# Autodesk Inventor assembly: Rover
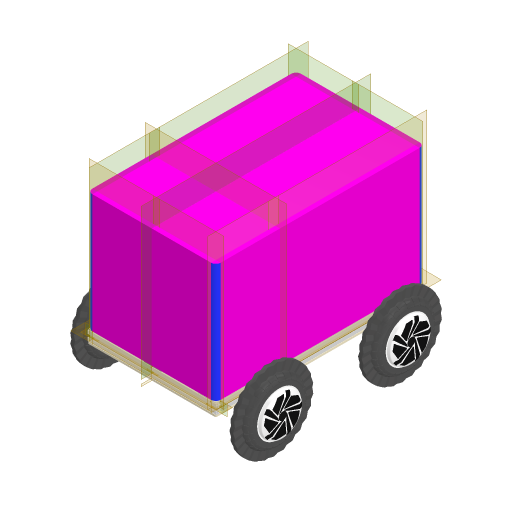
[picture p0: Inventor's stored thumbnail of the model, 512x512]
Saved by Autodesk Inventor 2023.2 (Build 272271030, 271C)
## iProperties
Created: 2024-10-30
Part Number: Rover
Document SubType Name: Assembly
Designer: I9232
Author: I9232
## Documents named in this file (10)
- D:\!Rover\Rover\Rover_construction\Rover.iam
- D:\!Rover\Rover\Rover_construction\platform.ipt
- D:\!Rover\Rover\Rover_construction\Motor, BLDC, Hoverboard Wheel, 8.0in.ipt
- D:\!Rover\Rover\Rover_construction\Profil 20x20.ipt
- D:\!Rover\Rover\Rover_construction\Крепление мотора.iam
- D:\!Rover\Rover\Rover_construction\Copter.ipt
- D:\!Rover\Rover\Rover_construction\Korpus.ipt
- D:\!Rover\Rover\Rover_construction\Уголок для профиля.ipt
- D:\!Rover\Rover\Rover_construction\Профиль 30x30\Профиль 30x30.ipt
- D:\!Rover\Rover\Rover_construction\Т-образный соединитель\Т-образный соединитель.ipt
## Components (33 placed, 10 different names)
1. platform:1 — Совмещение:1, Совмещение:2, Совмещение:107, Совмещение:119, Совмещение:120, Совмещение:121, Совмещение:169, Заподлицо:1, Заподлицо:2, Совмещение:170, Совмещение:171, Совмещение:172, Заподлицо:3, Заподлицо:4, Заподлицо:5, Заподлицо:6, Совмещение:180, Заподлицо:11
2. Copter:1
3. Корпус:1 — Совмещение:168
4. Profil 20x20:4 — Совмещение:149, Совмещение:167
5. Profil 20x20:5 — Совмещение:151, Совмещение:166
6. Profil 20x20:6 — Совмещение:152, Совмещение:165
7. Profil 20x20:7 — Совмещение:154, Совмещение:164
8. Profil 20x20:8 — Совмещение:150, Совмещение:166
9. Profil 20x20:9 — Совмещение:148, Совмещение:167
10. Profil 20x20:10 — Совмещение:153, Совмещение:165
11. Profil 20x20:11 — Совмещение:155, Совмещение:164
12. Т-образный соединитель:1 — Заподлицо:21, Совмещение:186, Совмещение:188
13. Т-образный соединитель:2 — Заподлицо:22, Совмещение:187, Заподлицо:23
14. Мотор гироскутера — Совмещение:122, Совмещение:123, Совмещение:124
15. Motor, BLDC, Hoverboard Wheel, 8.0in:4 — Совмещение:116, Совмещение:117, Совмещение:118
16. Motor, BLDC, Hoverboard Wheel, 8.0in:5 — Совмещение:112, Совмещение:113, Совмещение:115
17. Motor, BLDC, Hoverboard Wheel, 8.0in:6 — Совмещение:110, Совмещение:111, Совмещение:114
18. Profil 20x20:1 — Симметрия:3, Заподлицо:14, Совмещение:184, Заподлицо:18, Совмещение:185
19. Profil 20x20:2 — Симметрия:3, Заподлицо:12, Совмещение:181, Заподлицо:13, Заподлицо:20
20. Profil 20x20:3 — Заподлицо:18
21. Профиль 30x30:5 — Совмещение:179, Совмещение:180, Заподлицо:11, Заподлицо:21, Заподлицо:23
22. Профиль 30x30:2 — Совмещение:171, Совмещение:173, Заподлицо:3, Заподлицо:7, Заподлицо:10, Заподлицо:12, Совмещение:181, Совмещение:182, Совмещение:183
23. Профиль 30x30:3 — Совмещение:170, Заподлицо:5, Заподлицо:6, Совмещение:175, Совмещение:176, Совмещение:186, Совмещение:188
24. Профиль 30x30:4 — Совмещение:172, Совмещение:174, Заподлицо:4, Совмещение:177, Совмещение:178, Заподлицо:13, Заподлицо:14, Совмещение:184, Заподлицо:17, Заподлицо:19
25. Профиль 30x30:1 — Совмещение:169, Заподлицо:1, Заподлицо:2, Совмещение:173, Совмещение:174, Заподлицо:8, Заподлицо:9, Совмещение:179, Заподлицо:22, Совмещение:187
26. Крепление мотора:1 [sub-assembly] — Совмещение:116, Совмещение:117, Совмещение:118, Совмещение:119, Симметрия:2, Совмещение:152, Совмещение:153, Совмещение:183
27. Крепление мотора:2 [sub-assembly] — Совмещение:107, Совмещение:122, Совмещение:123, Совмещение:124, Симметрия:2, Совмещение:150, Совмещение:151, Заподлицо:19, Совмещение:185
28. Крепление мотора:3 [sub-assembly] — Совмещение:110, Совмещение:111, Совмещение:114, Совмещение:121, Симметрия:1, Совмещение:154, Совмещение:155, Совмещение:182, Заподлицо:20
29. Крепление мотора:4 [sub-assembly] — Совмещение:112, Совмещение:113, Совмещение:115, Совмещение:120, Симметрия:1, Совмещение:148, Совмещение:149, Заподлицо:17
30. Уголок для профиля:1 — Заподлицо:8, Совмещение:178
31. Уголок для профиля:2 — Совмещение:175, Заподлицо:7
32. Уголок для профиля:3 — Совмещение:168, Заподлицо:9, Заподлицо:10
33. Уголок для профиля:4 — Совмещение:176, Совмещение:177
## Relationships (75: Mate 51, Flush 21, Symmetry 3)
- Совмещение:1 [Mate]: platform:1
- Совмещение:2 [Mate]: platform:1
- Совмещение:107 [Mate]: platform:1 ↔ Крепление мотора:2
- Совмещение:110 [Mate]: Motor, BLDC, Hoverboard Wheel, 8.0in:6 ↔ Крепление мотора:3
- Совмещение:111 [Mate]: Motor, BLDC, Hoverboard Wheel, 8.0in:6 ↔ Крепление мотора:3
- Совмещение:112 [Mate]: Motor, BLDC, Hoverboard Wheel, 8.0in:5 ↔ Крепление мотора:4
- Совмещение:113 [Mate]: Motor, BLDC, Hoverboard Wheel, 8.0in:5 ↔ Крепление мотора:4
- Совмещение:114 [Mate]: Motor, BLDC, Hoverboard Wheel, 8.0in:6 ↔ Крепление мотора:3
- Совмещение:115 [Mate]: Motor, BLDC, Hoverboard Wheel, 8.0in:5 ↔ Крепление мотора:4
- Совмещение:116 [Mate]: Motor, BLDC, Hoverboard Wheel, 8.0in:4 ↔ Крепление мотора:1
- Совмещение:117 [Mate]: Motor, BLDC, Hoverboard Wheel, 8.0in:4 ↔ Крепление мотора:1
- Совмещение:118 [Mate]: Motor, BLDC, Hoverboard Wheel, 8.0in:4 ↔ Крепление мотора:1
- Совмещение:119 [Mate]: platform:1 ↔ Крепление мотора:1
- Совмещение:120 [Mate]: platform:1 ↔ Крепление мотора:4
- Совмещение:121 [Mate]: platform:1 ↔ Крепление мотора:3
- Совмещение:122 [Mate]: Мотор гироскутера ↔ Крепление мотора:2
- Совмещение:123 [Mate]: Мотор гироскутера ↔ Крепление мотора:2
- Совмещение:124 [Mate]: Мотор гироскутера ↔ Крепление мотора:2
- Симметрия:1 [Symmetry]: Крепление мотора:3 ↔ Крепление мотора:4
- Симметрия:2 [Symmetry]: Крепление мотора:1 ↔ Крепление мотора:2
- Симметрия:3 [Symmetry]: Profil 20x20:1 ↔ Profil 20x20:2
- Совмещение:148 [Mate]: Profil 20x20:9 ↔ Крепление мотора:4
- Совмещение:149 [Mate]: Profil 20x20:4 ↔ Крепление мотора:4
- Совмещение:150 [Mate]: Profil 20x20:8 ↔ Крепление мотора:2
- Совмещение:151 [Mate]: Profil 20x20:5 ↔ Крепление мотора:2
- Совмещение:152 [Mate]: Profil 20x20:6 ↔ Крепление мотора:1
- Совмещение:153 [Mate]: Profil 20x20:10 ↔ Крепление мотора:1
- Совмещение:154 [Mate]: Profil 20x20:7 ↔ Крепление мотора:3
- Совмещение:155 [Mate]: Profil 20x20:11 ↔ Крепление мотора:3
- Совмещение:164 [Mate] (30 mm): Profil 20x20:7 ↔ Profil 20x20:11
- Совмещение:165 [Mate] (30 mm): Profil 20x20:6 ↔ Profil 20x20:10
- Совмещение:166 [Mate] (30 mm): Profil 20x20:5 ↔ Profil 20x20:8
- Совмещение:167 [Mate] (30 mm): Profil 20x20:4 ↔ Profil 20x20:9
- Совмещение:168 [Mate]: Корпус:1 ↔ Уголок для профиля:3
- Совмещение:169 [Mate]: platform:1 ↔ Профиль 30x30:1
- Заподлицо:1 [Flush]: platform:1 ↔ Профиль 30x30:1
- Заподлицо:2 [Flush]: platform:1 ↔ Профиль 30x30:1
- Совмещение:170 [Mate]: platform:1 ↔ Профиль 30x30:3
- Совмещение:171 [Mate]: platform:1 ↔ Профиль 30x30:2
- Совмещение:172 [Mate]: platform:1 ↔ Профиль 30x30:4
- Совмещение:173 [Mate]: Профиль 30x30:2 ↔ Профиль 30x30:1
- Заподлицо:3 [Flush]: platform:1 ↔ Профиль 30x30:2
- Совмещение:174 [Mate]: Профиль 30x30:4 ↔ Профиль 30x30:1
- Заподлицо:4 [Flush]: platform:1 ↔ Профиль 30x30:4
- Заподлицо:5 [Flush]: platform:1 ↔ Профиль 30x30:3
- Заподлицо:6 [Flush]: platform:1 ↔ Профиль 30x30:3
- Совмещение:175 [Mate]: Профиль 30x30:3 ↔ Уголок для профиля:2
- Заподлицо:7 [Flush]: Профиль 30x30:2 ↔ Уголок для профиля:2
- Совмещение:176 [Mate]: Профиль 30x30:3 ↔ Уголок для профиля:4
- Совмещение:177 [Mate]: Профиль 30x30:4 ↔ Уголок для профиля:4
- Заподлицо:8 [Flush]: Профиль 30x30:1 ↔ Уголок для профиля:1
- Совмещение:178 [Mate]: Профиль 30x30:4 ↔ Уголок для профиля:1
- Заподлицо:9 [Flush]: Профиль 30x30:1 ↔ Уголок для профиля:3
- Заподлицо:10 [Flush]: Профиль 30x30:2 ↔ Уголок для профиля:3
- Совмещение:179 [Mate]: Профиль 30x30:5 ↔ Профиль 30x30:1
- Совмещение:180 [Mate]: platform:1 ↔ Профиль 30x30:5
- Заподлицо:11 [Flush]: platform:1 ↔ Профиль 30x30:5
- Заподлицо:12 [Flush]: Profil 20x20:2 ↔ Профиль 30x30:2
- Совмещение:181 [Mate]: Profil 20x20:2 ↔ Профиль 30x30:2
- Заподлицо:13 [Flush]: Profil 20x20:2 ↔ Профиль 30x30:4
- Совмещение:182 [Mate]: Профиль 30x30:2 ↔ Крепление мотора:3
- Совмещение:183 [Mate]: Профиль 30x30:2 ↔ Крепление мотора:1
- Заподлицо:14 [Flush]: Profil 20x20:1 ↔ Профиль 30x30:4
- Совмещение:184 [Mate]: Profil 20x20:1 ↔ Профиль 30x30:4
- Заподлицо:17 [Flush]: Профиль 30x30:4 ↔ Крепление мотора:4
- Заподлицо:18 [Flush] (-200 mm): Profil 20x20:1 ↔ Profil 20x20:3
- Заподлицо:19 [Flush]: Профиль 30x30:4 ↔ Крепление мотора:2
- Совмещение:185 [Mate]: Profil 20x20:1 ↔ Крепление мотора:2
- Заподлицо:20 [Flush]: Profil 20x20:2 ↔ Крепление мотора:3
- Заподлицо:21 [Flush]: Т-образный соединитель:1 ↔ Профиль 30x30:5
- Совмещение:186 [Mate]: Т-образный соединитель:1 ↔ Профиль 30x30:3
- Заподлицо:22 [Flush]: Т-образный соединитель:2 ↔ Профиль 30x30:1
- Совмещение:187 [Mate]: Т-образный соединитель:2 ↔ Профиль 30x30:1
- Заподлицо:23 [Flush]: Т-образный соединитель:2 ↔ Профиль 30x30:5
- Совмещение:188 [Mate]: Т-образный соединитель:1 ↔ Профиль 30x30:3
